# Autodesk Inventor assembly: Full Body v1
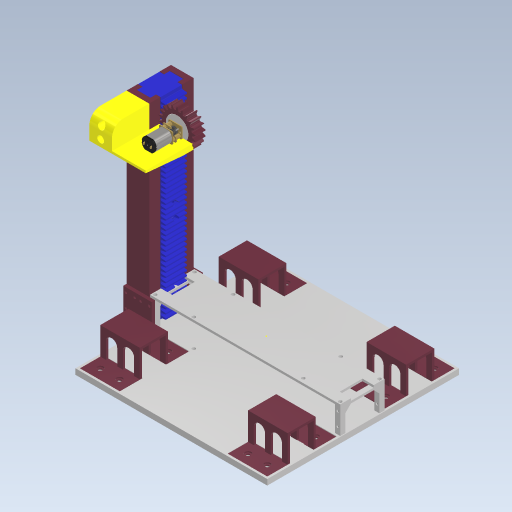
[picture p0: Inventor's stored thumbnail of the model, 512x512]
Saved by Autodesk Inventor 2023.5 (Build 275446000, 446)
## iProperties
Created: 2025-09-05
Part Number: Full Body v1
Document SubType Name: Assembly
Designer: Guntur
Author: Guntur
## Documents named in this file (12)
- F:\EEJ2025\design\Full Body v1.iam
- F:\EEJ2025\design\Casis.ipt
- F:\EEJ2025\design\Bracket Motor.ipt
- F:\EEJ2025\design\Tiang 1.ipt
- F:\EEJ2025\design\Casis Tengah.ipt
- F:\EEJ2025\design\Tiang Lifter.ipt
- F:\EEJ2025\design\Konektor Lifter.ipt
- F:\EEJ2025\design\Rack Lifter 2.ipt
- F:\EEJ2025\design\Holder Motor Lifter 2.ipt
- F:\EEJ2025\design\GearMotor\Motor.iam
- F:\EEJ2025\design\As Lifter.ipt
- F:\EEJ2025\design\Pinion Lifter.ipt
## Components (17 placed, 11 different names)
1. Casis:1 — Mate:1, Flush:1, Mate:2, Flush:2, Mate:3, Mate:4, Flush:3, Mate:5, Mate:6, Flush:4, Mate:7, Mate:8, Mate:9, Mate:10, Mate:11, Mate:12
2. Bracket Motor:1 — Flush:4, Mate:7, Mate:8
3. Bracket Motor:2 — Flush:3, Mate:5, Mate:6
4. Bracket Motor:3 — Flush:2, Mate:3, Mate:4
5. Bracket Motor:4 — Mate:1, Flush:1, Mate:2
6. Tiang 1:1 — Mate:9, Mate:10, Flush:5, Mate:23, Mate:24
7. Tiang 1:3 — Mate:11, Mate:12, Mate:15, Mate:16, Mate:19, Mate:20
8. Konektor Lifter:1 — Mate:15, Mate:16, Mate:17, Mate:18
9. Tiang Lifter:1 — Mate:17, Mate:18, Mate:25, Flush:6, Mate:31, Mate:32, Mate:33
10. Tiang Lifter:2 — Mate:21, Mate:22
11. Konektor Lifter:2 — Mate:19, Mate:20, Mate:21, Mate:22
12. Casis Tengah:1 — Flush:5, Mate:23, Mate:24
13. Rack Lifter 2:1 — Mate:25, Flush:6
14. GearMotor:1 [sub-assembly] — Mate:34, Mate:35, Flush:7
15. Holder Motor Lifter 2:1 — Mate:31, Mate:32, Mate:33, Mate:34
16. As Lifter:1 — Mate:35, Flush:7, Mate:36, Mate:37, Flush:8
17. Pinion Lifter:1 — Mate:36, Mate:37, Flush:8
## Relationships (38: Mate 30, Flush 8)
- Mate:1: Casis:1 ↔ Bracket Motor:4
- Flush:1: Casis:1 ↔ Bracket Motor:4
- Mate:2: Casis:1 ↔ Bracket Motor:4
- Flush:2: Casis:1 ↔ Bracket Motor:3
- Mate:3: Casis:1 ↔ Bracket Motor:3
- Mate:4: Casis:1 ↔ Bracket Motor:3
- Flush:3: Casis:1 ↔ Bracket Motor:2
- Mate:5: Casis:1 ↔ Bracket Motor:2
- Mate:6: Casis:1 ↔ Bracket Motor:2
- Flush:4: Casis:1 ↔ Bracket Motor:1
- Mate:7: Casis:1 ↔ Bracket Motor:1
- Mate:8: Casis:1 ↔ Bracket Motor:1
- Mate:9: Casis:1 ↔ Tiang 1:1
- Mate:10: Casis:1 ↔ Tiang 1:1
- Mate:11: Casis:1 ↔ Tiang 1:3
- Mate:12: Casis:1 ↔ Tiang 1:3
- Mate:15: Tiang 1:3 ↔ Konektor Lifter:1
- Mate:16: Tiang 1:3 ↔ Konektor Lifter:1
- Mate:17: Konektor Lifter:1 ↔ Tiang Lifter:1
- Mate:18: Konektor Lifter:1 ↔ Tiang Lifter:1
- Mate:19: Tiang 1:3 ↔ Konektor Lifter:2
- Mate:20: Tiang 1:3 ↔ Konektor Lifter:2
- Mate:21: Tiang Lifter:2 ↔ Konektor Lifter:2
- Mate:22: Tiang Lifter:2 ↔ Konektor Lifter:2
- Flush:5: Tiang 1:1 ↔ Casis Tengah:1
- Mate:23: Tiang 1:1 ↔ Casis Tengah:1
- Mate:24: Tiang 1:1 ↔ Casis Tengah:1
- Mate:25 (0.15 mm): Tiang Lifter:1 ↔ Rack Lifter 2:1
- Flush:6: Tiang Lifter:1 ↔ Rack Lifter 2:1
- Mate:31: Tiang Lifter:1 ↔ Holder Motor Lifter 2:1
- Mate:32: Tiang Lifter:1 ↔ Holder Motor Lifter 2:1
- Mate:33: Tiang Lifter:1 ↔ Holder Motor Lifter 2:1
- Mate:34: GearMotor:1 ↔ Holder Motor Lifter 2:1
- Mate:35: GearMotor:1 ↔ As Lifter:1
- Flush:7: GearMotor:1 ↔ As Lifter:1
- Mate:36: As Lifter:1 ↔ Pinion Lifter:1
- Mate:37: As Lifter:1 ↔ Pinion Lifter:1
- Flush:8: As Lifter:1 ↔ Pinion Lifter:1
